# Autodesk Inventor assembly: Old_Idler_28
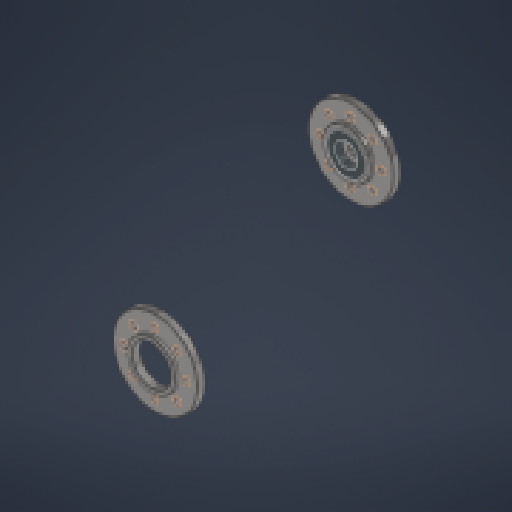
[picture p0: Inventor's stored thumbnail of the model, 512x512]
Saved by Autodesk Inventor 2024 (Build 280153000, 153)
## iProperties
Created: 2024-01-19
Part Number: Old_Idler_28
Document SubType Name: Assembly
Designer: ASUS
Author: ASUS
## Documents named in this file (4)
- C:\Users\ASUS\Desktop\2024_Robit_Hardware\ROBOCUP_2024_eindhoven\ROBOTIS(Inventor 2023 ver.)\아이들러\Old_Idler_28.iam
- C:\Users\ASUS\Desktop\2024_Robit_Hardware\ROBOCUP_2024_eindhoven\ROBOTIS(Inventor 2023 ver.)\아이들러\MF106ZZ.ipt
- C:\Users\ASUS\Desktop\2024_Robit_Hardware\ROBOCUP_2024_eindhoven\ROBOTIS(Inventor 2023 ver.)\아이들러\RX28-CAP.ipt
- C:\Users\ASUS\Desktop\2024_Robit_Hardware\ROBOCUP_2024_eindhoven\ROBOTIS(Inventor 2023 ver.)\아이들러\HN07-i101_Old.ipt
## Components (3 placed, 3 different names)
1. MF106ZZ:1 — 메이트:1, 메이트:2
2. RX28-CAP:1
3. HN07-i101_Old:2 — 메이트:1, 메이트:2
## Relationships (3: Mate 2, Insert 1)
- [Insert]: MF106ZZ:1 ↔ RX28-CAP:1
- 메이트:1 [Mate]: MF106ZZ:1 ↔ HN07-i101_Old:2
- 메이트:2 [Mate]: MF106ZZ:1 ↔ HN07-i101_Old:2
## Named parameters: d0_d1 = 0 mm
